# Autodesk Inventor assembly: battery_tube
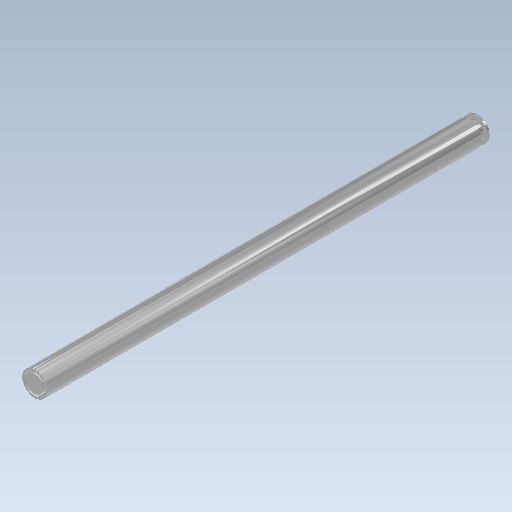
[picture p0: Inventor's stored thumbnail of the model, 512x512]
Saved by Autodesk Inventor 2020 (Build 240168000, 168)
## iProperties
Created: 2016-11-18
Part Number: battery_tube
Document SubType Name: Assembly
Designer: jous
Mass: 503.544 g
Surface Area: 2883.43 cm^2
Volume: 503.544 cm^3
Density: 1 g/cm^3
Author: jous
## Documents named in this file (4)
- C:\Users\jous\Desktop\boat\battery_tube.iam
- C:\Users\jous\Desktop\boat\battery_tube.ipt
- C:\Users\jous\Desktop\boat\battery_cap.ipt
- C:\Users\jous\Desktop\boat\battery_endcap.ipt
## Components (3 placed, 3 different names)
1. battery_tube:1 — Rigid:2, Rigid:1
2. battery_cap:2 — Rigid:2
3. battery_endcap:1 — Rigid:1
## Relationships (2: WeldJoint 2)
- Rigid:2 [WeldJoint]: battery_tube:1 ↔ battery_cap:2
- Rigid:1 [WeldJoint]: battery_tube:1 ↔ battery_endcap:1
